# Autodesk Inventor assembly: ヘルツ応力解析
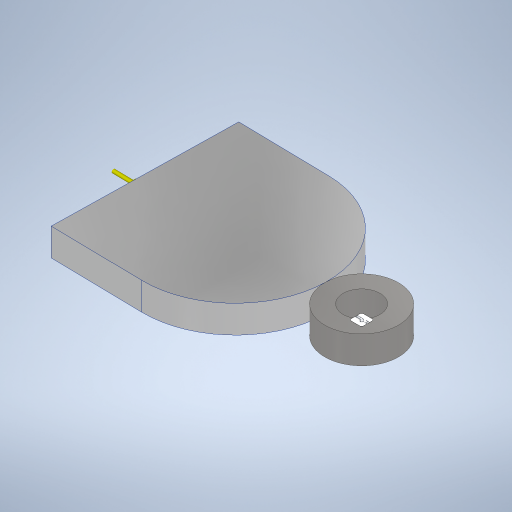
[picture p0: Inventor's stored thumbnail of the model, 512x512]
Saved by Autodesk Inventor 2024 (Build 280153000, 153)
## iProperties
Created: 2023-05-31
Part Number: ヘルツ応力解析
Document SubType Name: Assembly
Designer: yuta2
Author: yuta2
## Documents named in this file (9)
- C:\Users\yuta2\Documents\Inventor\mokemoke2023\サイクロイド減速機_大型\ヘルツ応力解析.iam
- C:\Users\yuta2\Documents\Inventor\mokemoke2023\サイクロイド減速機_大型\ベアリング想定.ipt
- C:\Users\yuta2\Documents\Inventor\mokemoke2023\サイクロイド減速機_大型\サイクロイドギア想定.ipt
- C:\Users\yuta2\Documents\Inventor\mokemoke2023\サイクロイド減速機_大型\ヘルツ応力解析\AIP\FEA\eco8pm0bk.fins
- C:\Users\yuta2\Documents\Inventor\mokemoke2023\サイクロイド減速機_大型\ヘルツ応力解析\AIP\FEA\eco8pm0cg.fsat
- C:\Users\yuta2\Documents\Inventor\mokemoke2023\サイクロイド減速機_大型\ヘルツ応力解析\AIP\FEA\eco8pm0cg.ftes
- C:\Users\yuta2\Documents\Inventor\mokemoke2023\サイクロイド減速機_大型\ヘルツ応力解析\AIP\FEA\eco8pm0cg.fwiz
- C:\Users\yuta2\Documents\Inventor\mokemoke2023\サイクロイド減速機_大型\ヘルツ応力解析\AIP\FEA\eco8pm0io.fmsh
- C:\Users\yuta2\Documents\Inventor\mokemoke2023\サイクロイド減速機_大型\ヘルツ応力解析\AIP\FEA\eco8pm0jk.fres
## Components (2 placed, 2 different names)
1. ベアリング想定:1 — フラッシュ:1, 正接:1, 正接:2
2. サイクロイドギア想定:1 — フラッシュ:1, 正接:1, 正接:2
## Relationships (3: Tangent 2, Flush 1)
- フラッシュ:1 [Flush]: ベアリング想定:1 ↔ サイクロイドギア想定:1
- 正接:1 [Tangent] (6 mm): ベアリング想定:1 ↔ サイクロイドギア想定:1
- 正接:2 [Tangent]: ベアリング想定:1 ↔ サイクロイドギア想定:1
## Named parameters: sa_0 = 45000
note: some values were not read from the file. Shown as the stored number, unit unknown: "sa_0".
